# Autodesk Inventor assembly: Akku
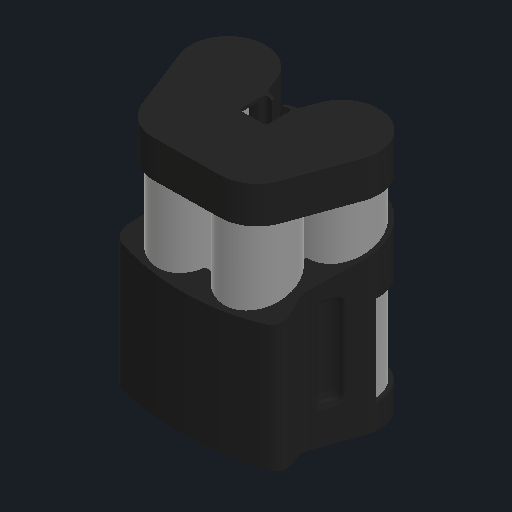
[picture p0: Inventor's stored thumbnail of the model, 512x512]
Saved by Autodesk Inventor 2025.2 (Build 292293000, 293)
## iProperties
Created: 2024-05-16
Part Number: Akku
Document SubType Name: Assembly
Designer: Fabian
Author: Fabian
## Documents named in this file (4)
- C:\Users\Faabs\Desktop\HBG v2025\Oberbaugruppen\OBG-Akku\OBG-Akku.iam
- C:\Users\Faabs\Desktop\HBG v2025\Oberbaugruppen\OBG-Akku\Bauteile\Halterung.ipt
- C:\Users\Faabs\Desktop\HBG v2025\Oberbaugruppen\OBG-Akku\Bauteile\Li-Io Zelle.ipt
- C:\Users\Faabs\Desktop\HBG v2025\Oberbaugruppen\OBG-Akku\Bauteile\Abdeckung.ipt
## Components (6 placed, 3 different names)
1. Halterung:1 — Passend:1, Passend:2, Passend:3, Passend:4, Passend:6, Passend:7, Passend:8, Passend:9
2. Li-Io Zelle:1 — Passend:4, Passend:9
3. Li-Io Zelle:2 — Passend:3, Passend:6, Passend:12
4. Li-Io Zelle:3 — Passend:1, Passend:8, Passend:11
5. Li-Io Zelle:4 — Passend:2, Passend:7, Passend:10
6. Abdeckung:1 — Passend:10, Passend:11, Passend:12
## Relationships (11: Mate 11)
- Passend:1 [Mate]: Halterung:1 ↔ Li-Io Zelle:3
- Passend:2 [Mate]: Halterung:1 ↔ Li-Io Zelle:4
- Passend:3 [Mate]: Halterung:1 ↔ Li-Io Zelle:2
- Passend:4 [Mate]: Halterung:1 ↔ Li-Io Zelle:1
- Passend:6 [Mate]: Halterung:1 ↔ Li-Io Zelle:2
- Passend:7 [Mate]: Halterung:1 ↔ Li-Io Zelle:4
- Passend:8 [Mate]: Halterung:1 ↔ Li-Io Zelle:3
- Passend:9 [Mate]: Halterung:1 ↔ Li-Io Zelle:1
- Passend:10 [Mate]: Li-Io Zelle:4 ↔ Abdeckung:1
- Passend:11 [Mate]: Li-Io Zelle:3 ↔ Abdeckung:1
- Passend:12 [Mate]: Li-Io Zelle:2 ↔ Abdeckung:1
